# Autodesk Inventor assembly: Sestava2
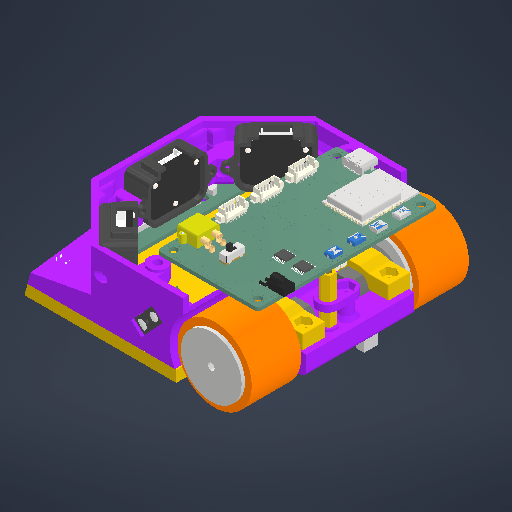
[picture p0: Inventor's stored thumbnail of the model, 512x512]
Saved by Autodesk Inventor 2025 (Build 290162000, 162)
## iProperties
Created: 2024-01-31
Part Number: Sestava2
Document SubType Name: Assembly
Designer: Simak
Author: Simak
## Documents named in this file (16)
- C:\_desktop\GitHub\Sumec-MiniSumo\-3D-\_wip\Sestava2.iam
- C:\_desktop\GitHub\Sumec-MiniSumo\-3D-\mech._parts\base_plate_v2.ipt
- C:\_desktop\GitHub\Sumec-MiniSumo\-3D-\PCBs\QRE MiniBoards\QRE MiniBoards\QRE_MiniBoards_Board.iam
- C:\_desktop\GitHub\Sumec-MiniSumo\-3D-\_wip\body.ipt
- C:\_desktop\GitHub\Sumec-MiniSumo\-3D-\mech._parts\box.ipt
- C:\_desktop\GitHub\Sumec-MiniSumo\-3D-\mech._parts\JSUMO_Wheel_33x25mm.ipt
- C:\_desktop\GitHub\Sumec-MiniSumo\-3D-\el._parts\3s lipo.ipt
- C:\_desktop\GitHub\Sumec-MiniSumo\-3D-\el._parts\2s lipo.ipt
- C:\_desktop\GitHub\Sumec-MiniSumo\-3D-\mech._parts\m3x20mm distanční sloupek.ipt
- C:\_desktop\GitHub\Sumec-MiniSumo\-3D-\_wip\TF-Luna_holder_v2\TF-Luna_holder_sestava_v2.iam
- C:\_desktop\GitHub\Sumec-MiniSumo\-3D-\el._parts\SensorSharpDigital\side_senzor.iam
- C:\_desktop\GitHub\Sumec-MiniSumo\-3D-\el._parts\qre_module_V2.ipt
- C:\_desktop\GitHub\Sumec-MiniSumo\-3D-\mech._parts\miniboard nutt holder.ipt
- C:\_desktop\GitHub\Sumec-MiniSumo\-3D-\mech._parts\motor_C_clamp_nutt_motor_otoceny.ipt
- C:\_desktop\GitHub\Sumec-MiniSumo\-3D-\el._parts\GA12-N20_Motor.ipt
- C:\_desktop\GitHub\Sumec-MiniSumo\-3D-\PCBs\main board\SUMEC_MK_IV.iam
## Components (19 placed, 15 different names)
1. base_plate_v2:1 — Proti sobě:3, Stejný směr:2, Vložit:1, Proti sobě:4, Stejný směr:3, Stejný směr:4, Proti sobě:7, Proti sobě:8, Proti sobě:9, Stejný směr:16
2. QRE_MiniBoards_Board:1 [sub-assembly] — Proti sobě:3, Stejný směr:2, Vložit:1, Proti sobě:30, Stejný směr:17, Vložit:10
3. body:1 — Proti sobě:4, Stejný směr:3, Stejný směr:4, Stejný směr:5, Stejný směr:6, Proti sobě:25, Proti sobě:26, Stejný směr:9, Stejný směr:10, Vložit:4, Vložit:6, Proti sobě:27, Vložit:7, Proti sobě:28, Stejný směr:14, Stejný směr:15, Proti sobě:31, Vložit:11, Stejný směr:18, Proti sobě:32, Stejný směr:19, Vložit:12, Proti sobě:33, Proti sobě:34, Vložit:13, Proti sobě:35, Proti sobě:36, Vložit:14, Proti sobě:37, Stejný směr:20
4. box:1 — Proti sobě:7, Proti sobě:8, Proti sobě:9, Proti sobě:10, Tečnost:1, Tečnost:2
5. JSUMO_Wheel_33x25mm:1 — Stejný směr:5, Proti sobě:11
6. JSUMO_Wheel_33x25mm:2 — Proti sobě:10, Tečnost:1, Tečnost:2, Proti sobě:11
7. 3s lipo:1
8. 2s lipo:1
9. m3x20mm distanční sloupek:1 — Stejný směr:6, Stejný směr:10, Vložit:4
10. TF-Luna_holder_sestava_v2:1 [sub-assembly] — Proti sobě:25, Proti sobě:26, Stejný směr:9
11. side_senzor:1 [sub-assembly] — Vložit:6, Proti sobě:27
12. side_senzor:2 [sub-assembly] — Vložit:7, Proti sobě:28
13. qre_module_V2:1 — Stejný směr:14, Stejný směr:15, Stejný směr:16
14. miniboard nutt holder:1 — Proti sobě:30, Stejný směr:17, Vložit:10
15. motor_C_clamp_nutt_motor_otoceny:1 — Proti sobě:32, Stejný směr:19, Vložit:12
16. motor_C_clamp_nutt_motor_otoceny:2 — Proti sobě:31, Vložit:11, Stejný směr:18
17. GA12-N20_Motor:1 — Proti sobě:35, Proti sobě:36, Vložit:14
18. GA12-N20_Motor:2 — Proti sobě:33, Proti sobě:34, Vložit:13
19. SUMEC_MK_IV:1 [sub-assembly] — Proti sobě:37, Stejný směr:20
## Relationships (44: Mate 19, Flush 14, Insert 9, Tangent 2)
- Proti sobě:3 [Mate] (1 mm): base_plate_v2:1 ↔ QRE_MiniBoards_Board:1
- Stejný směr:2 [Flush] (4.75 mm): base_plate_v2:1 ↔ QRE_MiniBoards_Board:1
- Vložit:1 [Insert]: base_plate_v2:1 ↔ QRE_MiniBoards_Board:1
- Proti sobě:4 [Mate]: base_plate_v2:1 ↔ body:1
- Stejný směr:3 [Flush]: base_plate_v2:1 ↔ body:1
- Stejný směr:4 [Flush]: base_plate_v2:1 ↔ body:1
- Proti sobě:7 [Mate] (2.5 mm): base_plate_v2:1 ↔ box:1
- Proti sobě:8 [Mate]: base_plate_v2:1 ↔ box:1
- Proti sobě:9 [Mate]: base_plate_v2:1 ↔ box:1
- Proti sobě:10 [Mate]: box:1 ↔ JSUMO_Wheel_33x25mm:2
- Tečnost:1 [Tangent]: box:1 ↔ JSUMO_Wheel_33x25mm:2
- Tečnost:2 [Tangent]: box:1 ↔ JSUMO_Wheel_33x25mm:2
- Stejný směr:5 [Flush]: body:1 ↔ JSUMO_Wheel_33x25mm:1
- Proti sobě:11 [Mate]: JSUMO_Wheel_33x25mm:1 ↔ JSUMO_Wheel_33x25mm:2
- Stejný směr:6 [Flush]: body:1 ↔ m3x20mm distanční sloupek:1
- Proti sobě:25 [Mate]: body:1 ↔ TF-Luna_holder_sestava_v2:1
- Proti sobě:26 [Mate]: body:1 ↔ TF-Luna_holder_sestava_v2:1
- Stejný směr:9 [Flush]: body:1 ↔ TF-Luna_holder_sestava_v2:1
- Stejný směr:10 [Flush]: body:1 ↔ m3x20mm distanční sloupek:1
- Vložit:4 [Insert]: body:1 ↔ m3x20mm distanční sloupek:1
- Vložit:6 [Insert]: body:1 ↔ side_senzor:1
- Proti sobě:27 [Mate]: body:1 ↔ side_senzor:1
- Vložit:7 [Insert]: body:1 ↔ side_senzor:2
- Proti sobě:28 [Mate]: body:1 ↔ side_senzor:2
- Stejný směr:14 [Flush]: body:1 ↔ qre_module_V2:1
- Stejný směr:15 [Flush]: body:1 ↔ qre_module_V2:1
- Stejný směr:16 [Flush] (-0.5 mm): base_plate_v2:1 ↔ qre_module_V2:1
- Proti sobě:30 [Mate]: QRE_MiniBoards_Board:1 ↔ miniboard nutt holder:1
- Stejný směr:17 [Flush]: QRE_MiniBoards_Board:1 ↔ miniboard nutt holder:1
- Vložit:10 [Insert]: QRE_MiniBoards_Board:1 ↔ miniboard nutt holder:1
- Proti sobě:31 [Mate] (1 mm): body:1 ↔ motor_C_clamp_nutt_motor_otoceny:2
- Vložit:11 [Insert]: body:1 ↔ motor_C_clamp_nutt_motor_otoceny:2
- Stejný směr:18 [Flush]: body:1 ↔ motor_C_clamp_nutt_motor_otoceny:2
- Proti sobě:32 [Mate] (1 mm): body:1 ↔ motor_C_clamp_nutt_motor_otoceny:1
- Stejný směr:19 [Flush]: body:1 ↔ motor_C_clamp_nutt_motor_otoceny:1
- Vložit:12 [Insert]: body:1 ↔ motor_C_clamp_nutt_motor_otoceny:1
- Proti sobě:33 [Mate]: body:1 ↔ GA12-N20_Motor:2
- Proti sobě:34 [Mate]: body:1 ↔ GA12-N20_Motor:2
- Vložit:13 [Insert]: body:1 ↔ GA12-N20_Motor:2
- Proti sobě:35 [Mate]: body:1 ↔ GA12-N20_Motor:1
- Proti sobě:36 [Mate]: body:1 ↔ GA12-N20_Motor:1
- Vložit:14 [Insert]: body:1 ↔ GA12-N20_Motor:1
- Proti sobě:37 [Mate]: body:1 ↔ SUMEC_MK_IV:1
- Stejný směr:20 [Flush]: body:1 ↔ SUMEC_MK_IV:1
## Named parameters: Finish1_Area = 2.15
note: some values were not read from the file. Shown as the stored number, unit unknown: "Finish1_Area".
